# Autodesk Inventor assembly: 5340825 CMMT-AS-C4-3A-EP-S1
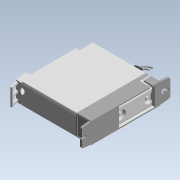
[picture p0: Inventor's stored thumbnail of the model, 180x180]
Saved by Autodesk Inventor 2021 (Build 250183000, 183)
## iProperties
Category: PARTsolutions
Company: FESTO
Part Number: 5340825 CMMT-AS-C4-3A-EP-S1
Catalog Web Link: www.cadenas.de
Description: CMMT-servo drive
Vendor: FESTO
Document SubType Name: Assembly
Designer: partserver
Manufacturer: FESTO
Mass: 1400 g
Surface Area: 1425.08 cm^2
Volume: 1409.13 cm^3
Density: 0.993519 g/cm^3
PSOL_IDENT_0: {ATYP=ASSISTANT},{DATA=script=$CADENAS_DATA/23d-libs/festo/webfesto.vbb&M_FAMILY=CMMT&M_GROUP=01&M_P
PSOL_IDENT_1: ARTNO=5340825&IDCODE1=CMMT-AS-C4-3A-EP-S1&IDCODE2=&customer_number_cns=&MATES=1&LOD=HI&LOCKERP=0&SIN
PSOL_IDENT_2: GLEPART=1}
NB: 5340825 CMMT-AS-C4-3A-EP-S1
NN: CMMT
NT: servo drive
NBSYN: $TNR. $TYP.
LINA: 5340825 CMMT-AS-C4-3A-EP-S1
CATALOG: Festo
TNR: 5340825
TYP: CMMT-AS-C4-3A-EP-S1
B1: 0
B2: 0
B3: 0
D1: 0
D2: 0
D3: 0
H1: 0
H2: 0
L1: 0
L2: 0
L3: 0
L4: 0
L5: 0
L6: 0
L7: 0
CNSMASSEXACT: 1.4
SUPPLIER: FESTO
ARTICLENO: 5340825 CMMT-AS-C4-3A-EP-S1
BOMINFO: 5340825 CMMT-AS-C4-3A-EP-S1
CREATOR: CADENAS GmbH
Title: 5340825 CMMT-AS-C4-3A-EP-S1
Author: Cadenas PARTsolutions
Comments: servo drive
## Documents named in this file (5)
- C:\Users\andre\Documents\GitHub\Dis.-Mecatronico-E6\inventor proyecto\Tablero\DriveAvance\PARTserver0202108230417182353949810e898ce\AIS2021\5340825 CMMT-AS-C4-3A-EP-S1.iam
- C:\Users\andre\Documents\GitHub\Dis.-Mecatronico-E6\inventor proyecto\Tablero\DriveAvance\PARTserver0202108230417182353949810e898ce\AIS2021\5340825 CMMT-AS-C4-3A-EP-S1---(h).ipt
- C:\Users\andre\Documents\GitHub\Dis.-Mecatronico-E6\inventor proyecto\Tablero\DriveAvance\PARTserver0202108230417182353949810e898ce\AIS2021\4978445 CMMT-AS-3A---(clamp).ipt
- C:\Users\andre\Documents\GitHub\Dis.-Mecatronico-E6\inventor proyecto\Tablero\DriveAvance\PARTserver0202108230417182353949810e898ce\AIS2021\ISO 14580 M4x16.ipt
- C:\Users\andre\Documents\GitHub\Dis.-Mecatronico-E6\inventor proyecto\Tablero\DriveAvance\PARTserver0202108230417182353949810e898ce\AIS2021\4021832 2GD-1RR7_62-CLP-CBL.ipt
## Components (5 placed, 4 different names)
1. 5340825 CMMT-AS-C4-3A-EP-S1---(h):1 — CLAMP_XY@1 <-> ANBAU_XY@3, CLAMP_Z@1 <-> ANBAU_Z@3, CLAMP_YZ@1 <-> ANBAU_YZ@3, PLUG_XY@1 <-> ANBAU_XY@6, PLUG_Z@1 <-> ANBAU_Z@6, PLUG_YZ@1 <-> ANBAU_YZ@6
2. 4978445 CMMT-AS-3A---(clamp):1 — CLAMP_XY@1 <-> ANBAU_XY@3, CLAMP_Z@1 <-> ANBAU_Z@3, CLAMP_YZ@1 <-> ANBAU_YZ@3, SCREW_1_XY@3 <-> IP1_XY@4, SCREW_1_Z@3 <-> IP1_Z@4, SCREW_1_YZ@3 <-> IP1_YZ@4, SCREW_2_XY@3 <-> IP1_XY@5, SCREW_2_Z@3 <-> IP1_Z@5, SCREW_2_YZ@3 <-> IP1_YZ@5
3. ISO 14580 M4x16:1 — SCREW_1_XY@3 <-> IP1_XY@4, SCREW_1_Z@3 <-> IP1_Z@4, SCREW_1_YZ@3 <-> IP1_YZ@4
4. ISO 14580 M4x16:2 — SCREW_2_XY@3 <-> IP1_XY@5, SCREW_2_Z@3 <-> IP1_Z@5, SCREW_2_YZ@3 <-> IP1_YZ@5
5. 4021832 2GD-1RR7_62-CLP-CBL:1 — PLUG_XY@1 <-> ANBAU_XY@6, PLUG_Z@1 <-> ANBAU_Z@6, PLUG_YZ@1 <-> ANBAU_YZ@6
## Relationships (12: Mate 8, Angle 4)
- CLAMP_XY@1 <-> ANBAU_XY@3 [Mate]: 5340825 CMMT-AS-C4-3A-EP-S1---(h):1 ↔ 4978445 CMMT-AS-3A---(clamp):1
- CLAMP_Z@1 <-> ANBAU_Z@3 [Mate]: 5340825 CMMT-AS-C4-3A-EP-S1---(h):1 ↔ 4978445 CMMT-AS-3A---(clamp):1
- CLAMP_YZ@1 <-> ANBAU_YZ@3 [Angle] (0 deg): 5340825 CMMT-AS-C4-3A-EP-S1---(h):1 ↔ 4978445 CMMT-AS-3A---(clamp):1
- SCREW_1_XY@3 <-> IP1_XY@4 [Mate]: 4978445 CMMT-AS-3A---(clamp):1 ↔ ISO 14580 M4x16:1
- SCREW_1_Z@3 <-> IP1_Z@4 [Mate]: 4978445 CMMT-AS-3A---(clamp):1 ↔ ISO 14580 M4x16:1
- SCREW_1_YZ@3 <-> IP1_YZ@4 [Angle] (0 deg): 4978445 CMMT-AS-3A---(clamp):1 ↔ ISO 14580 M4x16:1
- SCREW_2_XY@3 <-> IP1_XY@5 [Mate]: 4978445 CMMT-AS-3A---(clamp):1 ↔ ISO 14580 M4x16:2
- SCREW_2_Z@3 <-> IP1_Z@5 [Mate]: 4978445 CMMT-AS-3A---(clamp):1 ↔ ISO 14580 M4x16:2
- SCREW_2_YZ@3 <-> IP1_YZ@5 [Angle] (0 deg): 4978445 CMMT-AS-3A---(clamp):1 ↔ ISO 14580 M4x16:2
- PLUG_XY@1 <-> ANBAU_XY@6 [Mate]: 5340825 CMMT-AS-C4-3A-EP-S1---(h):1 ↔ 4021832 2GD-1RR7_62-CLP-CBL:1
- PLUG_Z@1 <-> ANBAU_Z@6 [Mate]: 5340825 CMMT-AS-C4-3A-EP-S1---(h):1 ↔ 4021832 2GD-1RR7_62-CLP-CBL:1
- PLUG_YZ@1 <-> ANBAU_YZ@6 [Angle] (0 deg): 5340825 CMMT-AS-C4-3A-EP-S1---(h):1 ↔ 4021832 2GD-1RR7_62-CLP-CBL:1
